# Autodesk Inventor assembly: クランク_MIR
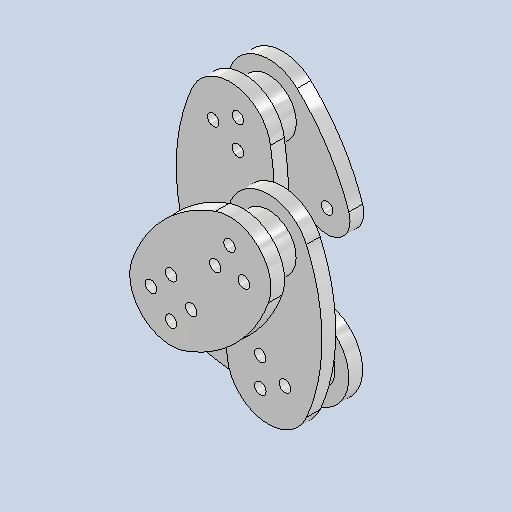
[picture p0: Inventor's stored thumbnail of the model, 512x512]
Saved by Autodesk Inventor 2023 (Build 270158000, 158)
## iProperties
Created: 2022-01-08
Part Number: クランク_MIR
Document SubType Name: Assembly
Designer: acps
Author: acps
## Documents named in this file (5)
- C:\Users\acps\Documents\srdc\srdc_ksh\脚\クランク_MIR.iam
- C:\Users\acps\Documents\srdc\srdc_ksh\カム\カム3_MIR.ipt
- C:\Users\acps\Documents\srdc\srdc_ksh\クランク\クランク_前_MIR.ipt
- C:\Users\acps\Documents\srdc\srdc_ksh\クランク\クランク_中間_MIR.ipt
- C:\Users\acps\Documents\srdc\srdc_ksh\クランク\駆動節_MIR.ipt
## Components (9 placed, 4 different names)
1. カム3_MIR:1 — Insert:9, Mate:18, Mate:17, Insert:2, Mate:4, Mate:3
2. カム3_MIR:2 — Insert:3, Mate:6, Mate:5, Insert:4, Mate:8, Mate:7
3. カム3_MIR:3 — Insert:10, Mate:10, Mate:9, Insert:6, Mate:12, Mate:11
4. クランク_前_MIR:1 — Insert:9, Mate:18, Mate:17
5. クランク_中間_MIR:1 — Insert:3, Mate:6, Mate:5, Insert:2, Mate:4, Mate:3
6. クランク_中間_MIR:2 — Insert:10, Mate:10, Mate:9, Insert:4, Mate:8, Mate:7
7. クランク_中間_MIR:3 — Insert:6, Mate:12, Mate:11, Insert:7, Mate:14, Mate:13
8. カム3_MIR:4 — Insert:7, Mate:14, Mate:13, Insert:8, Mate:16, Mate:15
9. 駆動節_MIR:1 — Insert:8, Mate:16, Mate:15
## Relationships (24: Mate 16, Insert 8)
- Insert:9: カム3_MIR:1 ↔ クランク_前_MIR:1
- Mate:18: カム3_MIR:1 ↔ クランク_前_MIR:1
- Mate:17: カム3_MIR:1 ↔ クランク_前_MIR:1
- Insert:3: カム3_MIR:2 ↔ クランク_中間_MIR:1
- Mate:6: カム3_MIR:2 ↔ クランク_中間_MIR:1
- Mate:5: カム3_MIR:2 ↔ クランク_中間_MIR:1
- Insert:2: カム3_MIR:1 ↔ クランク_中間_MIR:1
- Mate:4: カム3_MIR:1 ↔ クランク_中間_MIR:1
- Mate:3: カム3_MIR:1 ↔ クランク_中間_MIR:1
- Insert:10: カム3_MIR:3 ↔ クランク_中間_MIR:2
- Mate:10: カム3_MIR:3 ↔ クランク_中間_MIR:2
- Mate:9: カム3_MIR:3 ↔ クランク_中間_MIR:2
- Insert:4: カム3_MIR:2 ↔ クランク_中間_MIR:2
- Mate:8: カム3_MIR:2 ↔ クランク_中間_MIR:2
- Mate:7: カム3_MIR:2 ↔ クランク_中間_MIR:2
- Insert:6: カム3_MIR:3 ↔ クランク_中間_MIR:3
- Mate:12: カム3_MIR:3 ↔ クランク_中間_MIR:3
- Mate:11: カム3_MIR:3 ↔ クランク_中間_MIR:3
- Insert:7: クランク_中間_MIR:3 ↔ カム3_MIR:4
- Mate:14: クランク_中間_MIR:3 ↔ カム3_MIR:4
- Mate:13: クランク_中間_MIR:3 ↔ カム3_MIR:4
- Insert:8: カム3_MIR:4 ↔ 駆動節_MIR:1
- Mate:16: カム3_MIR:4 ↔ 駆動節_MIR:1
- Mate:15: カム3_MIR:4 ↔ 駆動節_MIR:1
